# Autodesk Inventor assembly: Trave a terra
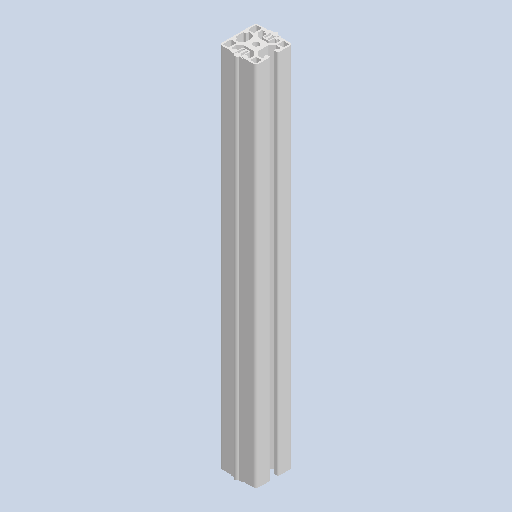
[picture p0: Inventor's stored thumbnail of the model, 512x512]
Saved by Autodesk Inventor 2022 (Build 260153000, 153)
## iProperties
RuleStatus: InUse
Created: 2022-01-26
Part Number: Trave a terra
Document SubType Name: Assembly
Designer: Elia
Author: Elia
## Documents named in this file (4)
- C:\Users\matte\Documents\GitHub\MDM-CyberOrto-CAD\Trave a terra\Trave a terra.iam
- C:\Users\matte\Documents\GitHub\MDM-CyberOrto-CAD\Nuova cartella (2)\pistaterra.ipt
- C:\Users\matte\Documents\GitHub\MDM-CyberOrto-CAD\Nuova cartella (2)\13-106.ipt
- C:\Users\matte\Documents\GitHub\MDM-CyberOrto-CAD\Nuova cartella (2)\13-513.ipt
## Components (5 placed, 3 different names)
1. pistaterra:1 — Coincidente:1, Coincidente:2, Coincidente:3, Coincidente:4, Allineato:1, Allineato:2
2. 13-106:1 — Coincidente:2, Coincidente:3, Allineato:1, Coincidente:5
3. 13-106:2 — Coincidente:1, Coincidente:4, Allineato:2, Coincidente:6
4. 13-513:1 — Coincidente:6
5. 13-513:2 — Coincidente:5
## Relationships (8: Mate 6, Flush 2)
- Coincidente:1 [Mate]: pistaterra:1 ↔ 13-106:2
- Coincidente:2 [Mate]: pistaterra:1 ↔ 13-106:1
- Coincidente:3 [Mate]: pistaterra:1 ↔ 13-106:1
- Coincidente:4 [Mate]: pistaterra:1 ↔ 13-106:2
- Allineato:1 [Flush]: pistaterra:1 ↔ 13-106:1
- Allineato:2 [Flush]: pistaterra:1 ↔ 13-106:2
- Coincidente:5 [Mate]: 13-106:1 ↔ 13-513:2
- Coincidente:6 [Mate]: 13-106:2 ↔ 13-513:1
